# Autodesk Inventor assembly: setNut
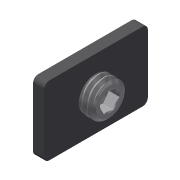
[picture p0: Inventor's stored thumbnail of the model, 180x180]
Saved by Autodesk Inventor 2017 (Build 210142000, 142)
## iProperties
Created: 2017-03-01
Part Number: setNut
Document SubType Name: Assembly
Designer: sawaiz
Author: sawaiz
## Documents named in this file (3)
- C:\Users\sawaiz\oneDrive\projects\sPhenixTileTestStand\hardware\setNut.iam
- C:\Users\sawaiz\oneDrive\projects\sPhenixTileTestStand\hardware\m5TNut.ipt
- C:\Users\sawaiz\oneDrive\projects\sPhenixTileTestStand\hardware\m5x6SetScrew.ipt
## Components (2 placed, 2 different names)
1. m5TNut:1 — Mate:1, Mate:2
2. m5x6SetScrew:1 — Mate:1, Mate:2
## Relationships (2: Mate 2)
- Mate:1: m5TNut:1 ↔ m5x6SetScrew:1
- Mate:2 (-4 mm): m5TNut:1 ↔ m5x6SetScrew:1
